# Autodesk Inventor assembly: 1.625 Flex, LS
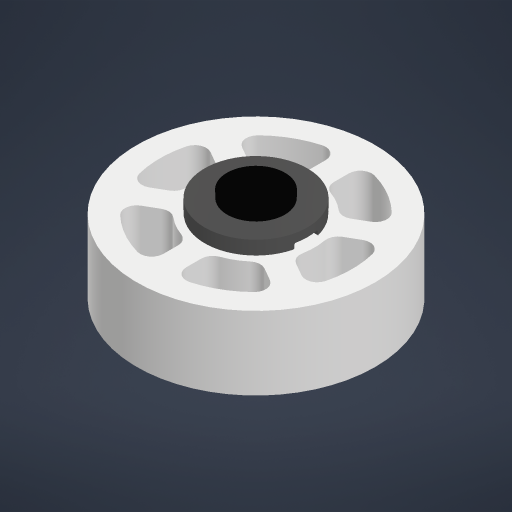
[picture p0: Inventor's stored thumbnail of the model, 512x512]
Saved by Autodesk Inventor 2023 (Build 270158000, 158)
## iProperties
Created: 2023-02-19
Part Number: 1.625 Flex, LS
Document SubType Name: Assembly
Designer: Windows Macbook
Author: Windows Macbook
## Documents named in this file (5)
- C:\Users\Windows Macbook\Desktop\Inventor\Motion\Wheels\Flex Wheels\1.625 Flex, LS.iam
- C:\Users\Windows Macbook\Desktop\Inventor\Motion\Wheels\Flex Wheels\1.625 Flex Wheel\1.625 30A .500.ipt
- C:\Users\Windows Macbook\Desktop\Inventor\Motion\Wheels\Flex Wheels\1.625 Flex Wheel.ipt
- C:\Users\Windows Macbook\Desktop\Inventor\Motion\Wheels\Flex Wheels\VersaHex Adapters .250.ipt
- C:\Users\Windows Macbook\Desktop\Inventor\Motion\Insert Square.ipt
## Components (5 placed, 3 different names)
1. 1.625 30A .500:1 — Insert:3, Angle:3, Insert:4
2. VersaHex Adapters .250:1 — Insert:3, Angle:3, Angle:4
3. Insert Square:1
4. VersaHex Adapters .250:2 — Angle:4, Insert:4
5. Insert Square:2
## Relationships (8: Insert 4, Angle 4)
- [Insert]: VersaHex Adapters .250:1 ↔ Insert Square:1
- [Angle] (0 deg): VersaHex Adapters .250:1 ↔ Insert Square:1
- [Insert]: VersaHex Adapters .250:2 ↔ Insert Square:2
- [Angle] (0 deg): VersaHex Adapters .250:2 ↔ Insert Square:2
- Insert:3: 1.625 30A .500:1 ↔ VersaHex Adapters .250:1
- Angle:3 (0 deg): 1.625 30A .500:1 ↔ VersaHex Adapters .250:1
- Angle:4 (0 deg): VersaHex Adapters .250:1 ↔ VersaHex Adapters .250:2
- Insert:4: 1.625 30A .500:1 ↔ VersaHex Adapters .250:2
## Named parameters: d2_d0 = 0 mm, d3_d1 = 0 deg
